# Autodesk Inventor assembly: chess
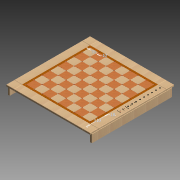
[picture p0: Inventor's stored thumbnail of the model, 180x180]
Saved by Autodesk Inventor 2013 SP1 (Build 170176100, 176)
## iProperties
Created: 2012-12-07
Part Number: chess
Document SubType Name: Assembly
Designer: Sebastian
Author: Sebastian
## Documents named in this file (12)
- E:\Projects\chess\construction\Schachcomputer.iam
- E:\Projects\chess\construction\Spielfeld.ipt
- E:\Projects\chess\construction\LED.ipt
- E:\Projects\chess\construction\Platine.ipt
- E:\Projects\chess\construction\Rahmen.ipt
- E:\Projects\chess\construction\Wände.ipt
- E:\Projects\chess\construction\Raspberry.ipt
- E:\Projects\chess\construction\Pushbutton.ipt
- E:\Projects\chess\construction\Schalterhalterung.ipt
- E:\Projects\chess\construction\Pin.ipt
- E:\Projects\chess\construction\Hohlstecker.ipt
- E:\Projects\chess\construction\RJ45-Buchse.ipt
## Components (138 placed, 11 different names)
1. Spielfeld:1 — Einfügen:4
2. Platine:1
3. Wände:1
4. Rahmen:1 — Einfügen:1, Einfügen:2, Einfügen:3
5. Raspberry:1
6. LED:82 — Einfügen:2
7. LED:83 — Einfügen:3
8. Schalterhalterung:1
9. Hohlstecker:1
10. RJ45-Buchse:1
11. LED:1 — Einfügen:4
12. LED:2
13. LED:3
14. LED:4
15. LED:5
16. LED:6
17. LED:7
18. LED:8
19. LED:9
20. LED:10
21. LED:11
22. LED:12
23. LED:13
24. LED:14
25. LED:15
26. LED:16
27. LED:17
28. LED:18
29. LED:19
30. LED:20
31. LED:21
32. LED:22
33. LED:23
34. LED:24
35. LED:25
36. LED:26
37. LED:27
38. LED:28
39. LED:29
40. LED:30
41. LED:31
42. LED:32
43. LED:33
44. LED:34
45. LED:35
46. LED:36
47. LED:37
48. LED:38
49. LED:39
50. LED:40
51. LED:41
52. LED:42
53. LED:43
54. LED:44
55. LED:45
56. LED:46
57. LED:47
58. LED:48
59. LED:49
60. LED:50
61. LED:51
62. LED:52
63. LED:53
64. LED:54
65. LED:55
66. LED:56
67. LED:57
68. LED:58
69. LED:59
70. LED:60
71. LED:61
72. LED:62
73. LED:63
74. LED:64
75. LED:65
76. LED:66
77. LED:67
78. LED:68
79. LED:69
80. LED:70
81. LED:71
82. LED:72
83. LED:73
84. LED:74
85. LED:75
86. LED:76
87. LED:77
88. LED:78
89. LED:79
90. LED:80
91. LED:81
92. Pushbutton:11 — Einfügen:1
93. Pushbutton:12
94. Pushbutton:13
95. Pushbutton:14
96. Pushbutton:15
97. Pushbutton:16
98. Pushbutton:17
99. Pushbutton:18
100. Pushbutton:19
101. Pin:1
102. Pin:2
103. Pin:3
104. Pin:4
105. Pin:5
106. Pin:6
107. Pin:7
108. Pin:8
109. Pin:9
110. Pin:10
111. Pin:11
112. Pin:12
113. Pin:13
114. Pin:14
115. Pin:15
116. Pin:16
117. Pin:17
118. Pin:18
119. Pin:19
120. Pin:20
121. Pin:21
122. Pin:22
123. Pin:23
124. Pin:24
125. Pin:25
126. Pin:26
127. Pin:27
128. Pin:28
129. Pin:29
130. Pin:30
131. Pin:31
132. Pin:32
133. Pin:33
134. Pin:34
135. Pin:35
136. Pin:36
137. Pin:37
138. Pin:38
## Component patterns: Komponentenanordnung LEDs (81 elements), Komponentenanordnung Schalter (9 elements), Komponentenanordnung Stiftleiste oben (13 elements), Komponentenanordnung Stiftleiste rechts (25 elements)
## Relationships (4: Insert 4)
- Einfügen:1 [Insert] (-10 mm): Rahmen:1 ↔ Pushbutton:11
- Einfügen:2 [Insert] (-6.5 mm): Rahmen:1 ↔ LED:82
- Einfügen:3 [Insert] (-6.5 mm): Rahmen:1 ↔ LED:83
- Einfügen:4 [Insert] (0.5 mm): Spielfeld:1 ↔ LED:1
